# Autodesk Inventor assembly: ROBOT-FINAL
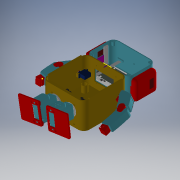
[picture p0: Inventor's stored thumbnail of the model, 180x180]
Saved by Autodesk Inventor 2019 (Build 230136000, 136)
## iProperties
Part Number: ROBOT-FINAL
Material: Genérico
Document SubType Name: Assembly
Designer: Kevin
Author: Kevin
## Documents named in this file (20)
- D:\Documents\Kevin\robot\ROBOT-FINAL.iam
- D:\Documents\Kevin\robot\CUERPO-VALIDO (1).ipt
- D:\Documents\Kevin\robot\EnsamblePierna.iam
- D:\Documents\Kevin\robot\brazo.iam
- D:\Documents\Kevin\robot\tapatronco.ipt
- D:\Documents\Kevin\robot\CABEZAFINAL.ipt
- C:\Users\flakt\Desktop\nuevacarpeta\rodamiento.ipt
- D:\Documents\Kevin\robot\servomotor-htx-900-1.snapshot.6\Servomotor HTX900.ipt
- D:\Documents\Kevin\robot\servomotor-htx-900-1.snapshot.6\Arm 1.ipt
- D:\Documents\Kevin\robot\brazos\brazoderech\tapatornillo.ipt
- D:\Documents\Kevin\robot\5inch-lcd-and-raspberry-pi-1.snapshot.1\5 inch LCD and PI\RPi3B+ and 5inch LCD.ipt
- D:\Documents\Kevin\robot\hitec-hsr-2645cr-1.snapshot.3\СЕРВА\03.ipt
- D:\Documents\Kevin\robot\Base.ipt
- D:\Documents\Kevin\robot\boton2.ipt
- D:\Documents\Kevin\robot\tapacuerpo.ipt
- D:\Documents\Kevin\robot\tapacabezaacrilico.ipt
- D:\Documents\Kevin\robot\botonrobotvero.ipt
- D:\Documents\Kevin\robot\piezaboton.ipt
- D:\Documents\Kevin\robot\piezasoportepantalla.ipt
- D:\Documents\Kevin\robot\soporte3pantalla.ipt
## Components (30 placed, 19 different names)
1. EnsamblePierna:1 [sub-assembly] — De rotación:2, De rotación:8
2. brazo:1 [sub-assembly] — De rotación:4, Rígido:14, Rígido:16
3. brazo:2 [sub-assembly] — De rotación:5, Rígido:12, Rígido:15
4. tapatronco:1 — Coincidencia:4
5. CABEZAFINAL:2 — Rígido:2, Rígido:3, Rígido:17, Rígido:21, Rígido:22, Rígido:24, Rígido:31, Rígido:32, De rotación:21, Rígido:36
6. rodamiento:1 — De rotación:17, De rotación:18
7. rodamiento:2 — De rotación:8, De rotación:16
8. Servomotor HTX900:1 — Rígido:4, De rotación:12
9. Servomotor HTX900:2 — Rígido:11, De rotación:11
10. Arm 1:1 — De rotación:12, Rígido:14
11. Arm 1:2 — De rotación:11, Rígido:12
12. tapatornillo:1 — Rígido:15
13. tapatornillo:2 — Rígido:16
14. RPi3B+ and 5inch LCD:1 — Rígido:17
15. 03:1 — De rotación:19
16. 03:2 — De rotación:20
17. Base:1 — Rígido:29, De rotación:19, De rotación:20
18. boton2:1 — Rígido:21
19. boton2:2 — Rígido:22
20. tapacuerpo:1 — Rígido:30
21. tapacabezaacrilico:1 — Rígido:24
22. EnsamblePierna:2 [sub-assembly] — De rotación:18
23. piezaboton:1 — Rígido:31
24. piezaboton:2 — Rígido:32
25. botonrobotvero:1 — Rígido:34
26. botonrobotvero:2 — Rígido:35
27. botonrobotvero:3 — Rígido:33
28. piezasoportepantalla:1 — De rotación:21
29. soporte3pantalla:1 — Rígido:36
30. CUERPO-VALIDO (1):1 — De rotación:2, De rotación:4, De rotación:5, Coincidencia:4, Rígido:2, Rígido:3, Rígido:11, Rígido:4, De rotación:16, De rotación:17, Rígido:29, Rígido:30, Rígido:33, Rígido:34, Rígido:35
## Relationships (33: WeldJoint 20, RevoluteJoint 12, Mate 1)
- De rotación:2 [RevoluteJoint] (-1 mm): EnsamblePierna:1 ↔ CUERPO-VALIDO (1):1
- De rotación:4 [RevoluteJoint] (-4 mm): brazo:1 ↔ CUERPO-VALIDO (1):1
- De rotación:5 [RevoluteJoint] (-4 mm): brazo:2 ↔ CUERPO-VALIDO (1):1
- Coincidencia:4 [Mate]: tapatronco:1 ↔ CUERPO-VALIDO (1):1
- De rotación:8 [RevoluteJoint] (-8 mm): EnsamblePierna:1 ↔ rodamiento:2
- Rígido:2 [WeldJoint]: CABEZAFINAL:2 ↔ CUERPO-VALIDO (1):1
- Rígido:3 [WeldJoint]: CABEZAFINAL:2 ↔ CUERPO-VALIDO (1):1
- Rígido:11 [WeldJoint]: Servomotor HTX900:2 ↔ CUERPO-VALIDO (1):1
- Rígido:4 [WeldJoint]: Servomotor HTX900:1 ↔ CUERPO-VALIDO (1):1
- De rotación:11 [RevoluteJoint]: Servomotor HTX900:2 ↔ Arm 1:2
- Rígido:12 [WeldJoint]: brazo:2 ↔ Arm 1:2
- De rotación:12 [RevoluteJoint]: Servomotor HTX900:1 ↔ Arm 1:1
- Rígido:14 [WeldJoint]: brazo:1 ↔ Arm 1:1
- Rígido:15 [WeldJoint]: brazo:2 ↔ tapatornillo:1
- Rígido:16 [WeldJoint]: brazo:1 ↔ tapatornillo:2
- Rígido:17 [WeldJoint]: CABEZAFINAL:2 ↔ RPi3B+ and 5inch LCD:1
- Rígido:21 [WeldJoint]: CABEZAFINAL:2 ↔ boton2:1
- Rígido:22 [WeldJoint]: CABEZAFINAL:2 ↔ boton2:2
- Rígido:24 [WeldJoint]: CABEZAFINAL:2 ↔ tapacabezaacrilico:1
- De rotación:16 [RevoluteJoint]: rodamiento:2 ↔ CUERPO-VALIDO (1):1
- De rotación:17 [RevoluteJoint]: rodamiento:1 ↔ CUERPO-VALIDO (1):1
- De rotación:18 [RevoluteJoint]: rodamiento:1 ↔ EnsamblePierna:2
- Rígido:29 [WeldJoint]: Base:1 ↔ CUERPO-VALIDO (1):1
- De rotación:19 [RevoluteJoint]: 03:1 ↔ Base:1
- De rotación:20 [RevoluteJoint]: 03:2 ↔ Base:1
- Rígido:30 [WeldJoint]: tapacuerpo:1 ↔ CUERPO-VALIDO (1):1
- Rígido:31 [WeldJoint]: CABEZAFINAL:2 ↔ piezaboton:1
- Rígido:32 [WeldJoint]: CABEZAFINAL:2 ↔ piezaboton:2
- Rígido:33 [WeldJoint]: botonrobotvero:3 ↔ CUERPO-VALIDO (1):1
- Rígido:34 [WeldJoint]: botonrobotvero:1 ↔ CUERPO-VALIDO (1):1
- Rígido:35 [WeldJoint]: botonrobotvero:2 ↔ CUERPO-VALIDO (1):1
- De rotación:21 [RevoluteJoint]: CABEZAFINAL:2 ↔ piezasoportepantalla:1
- Rígido:36 [WeldJoint]: CABEZAFINAL:2 ↔ soporte3pantalla:1
